# Autodesk Inventor assembly: 屋-2
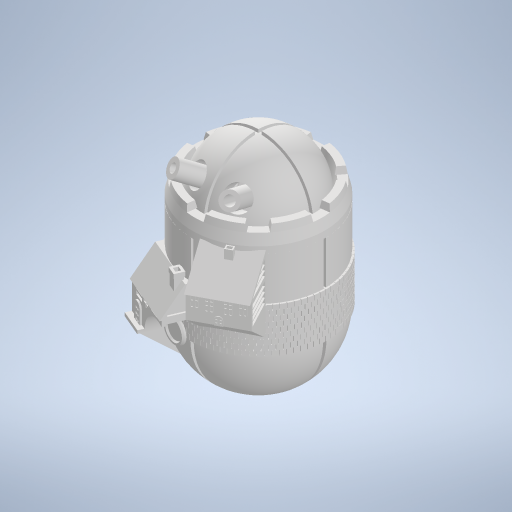
[picture p0: Inventor's stored thumbnail of the model, 512x512]
Saved by Autodesk Inventor 2024 (Build 280153000, 153)
## iProperties
Created: 2024-05-21
Part Number: 屋-2
Document SubType Name: Assembly
Designer: User
Author: User
## Documents named in this file (8)
- C:\Users\User\Documents\Inventor\construction\屋-2.iam
- C:\Users\User\Documents\Inventor\construction\屋頂-2.ipt
- C:\Users\User\Documents\Inventor\construction\屋-2 柱-1.ipt
- C:\Users\User\Documents\Inventor\construction\屋-2 磚-1.ipt
- C:\Users\User\Documents\Inventor\construction\屋-2 物1.ipt
- C:\Users\User\Documents\Inventor\construction\屋2 base.ipt
- C:\Users\User\Documents\Inventor\construction\屋2 物2.ipt
- C:\Users\User\Documents\Inventor\construction\屋2 孔1.ipt
## Components (15 placed, 7 different names)
1. 屋頂-2:1 — 貼合:1, 貼合:2
2. 屋-2 柱-1:1 — 貼合:1, 貼合:2, 貼合:3, 貼合:4, 貼合:6, 貼合:8, 貼合:10, 貼合:12, 貼合:14, 貼合:16, 貼合:18, 貼合:20, 貼合:24
3. 屋-2 磚-1:1 — 貼合:3, 貼合:4, 貼合:5, 貼合:22, 貼合:25
4. 屋-2 磚-1:2 — 貼合:5, 貼合:6, 貼合:7
5. 屋-2 磚-1:3 — 貼合:7, 貼合:8, 貼合:9
6. 屋-2 磚-1:4 — 貼合:11, 貼合:12, 貼合:13
7. 屋-2 磚-1:5 — 貼合:9, 貼合:10, 貼合:11
8. 屋-2 磚-1:6 — 貼合:13, 貼合:14, 貼合:15
9. 屋-2 磚-1:7 — 貼合:15, 貼合:16, 貼合:17
10. 屋-2 磚-1:8 — 貼合:19, 貼合:20, 貼合:23
11. 屋-2 磚-1:9 — 貼合:17, 貼合:18, 貼合:19, 貼合:26
12. 屋-2 物1:1 — 貼合:22
13. 屋2 base:1 — 貼合:23, 貼合:24
14. 屋2 物2:1 — 貼合:25
15. 屋2 孔1:1 — 貼合:26
## Relationships (25: Mate 25)
- 貼合:1 [Mate]: 屋頂-2:1 ↔ 屋-2 柱-1:1
- 貼合:2 [Mate]: 屋頂-2:1 ↔ 屋-2 柱-1:1
- 貼合:3 [Mate]: 屋-2 柱-1:1 ↔ 屋-2 磚-1:1
- 貼合:4 [Mate]: 屋-2 柱-1:1 ↔ 屋-2 磚-1:1
- 貼合:5 [Mate]: 屋-2 磚-1:1 ↔ 屋-2 磚-1:2
- 貼合:6 [Mate]: 屋-2 柱-1:1 ↔ 屋-2 磚-1:2
- 貼合:7 [Mate]: 屋-2 磚-1:2 ↔ 屋-2 磚-1:3
- 貼合:8 [Mate]: 屋-2 柱-1:1 ↔ 屋-2 磚-1:3
- 貼合:9 [Mate]: 屋-2 磚-1:3 ↔ 屋-2 磚-1:5
- 貼合:10 [Mate]: 屋-2 柱-1:1 ↔ 屋-2 磚-1:5
- 貼合:11 [Mate]: 屋-2 磚-1:4 ↔ 屋-2 磚-1:5
- 貼合:12 [Mate]: 屋-2 柱-1:1 ↔ 屋-2 磚-1:4
- 貼合:13 [Mate]: 屋-2 磚-1:4 ↔ 屋-2 磚-1:6
- 貼合:14 [Mate]: 屋-2 柱-1:1 ↔ 屋-2 磚-1:6
- 貼合:15 [Mate]: 屋-2 磚-1:6 ↔ 屋-2 磚-1:7
- 貼合:16 [Mate]: 屋-2 柱-1:1 ↔ 屋-2 磚-1:7
- 貼合:17 [Mate]: 屋-2 磚-1:7 ↔ 屋-2 磚-1:9
- 貼合:18 [Mate]: 屋-2 柱-1:1 ↔ 屋-2 磚-1:9
- 貼合:19 [Mate]: 屋-2 磚-1:8 ↔ 屋-2 磚-1:9
- 貼合:20 [Mate]: 屋-2 柱-1:1 ↔ 屋-2 磚-1:8
- 貼合:22 [Mate]: 屋-2 磚-1:1 ↔ 屋-2 物1:1
- 貼合:23 [Mate]: 屋-2 磚-1:8 ↔ 屋2 base:1
- 貼合:24 [Mate]: 屋-2 柱-1:1 ↔ 屋2 base:1
- 貼合:25 [Mate] (-16 mm): 屋-2 磚-1:1 ↔ 屋2 物2:1
- 貼合:26 [Mate]: 屋-2 磚-1:9 ↔ 屋2 孔1:1
